# Autodesk Inventor assembly: PeltierController
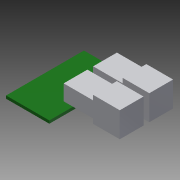
[picture p0: Inventor's stored thumbnail of the model, 180x180]
Saved by Autodesk Inventor 2014 (Build 180170000, 170)
## iProperties
Created: 2015-04-19
Part Number: PeltierController
Document SubType Name: Assembly
Designer: Owner
Author: Owner
## Documents named in this file (4)
- C:\Users\Owner\Documents\APC\FrontEnd\IAM\Common\PeltierController.iam
- C:\Users\Owner\Documents\APC\FrontEnd\IAM\Common\PeltierControllerBoard.ipt
- C:\Users\Owner\Documents\APC\FrontEnd\IAM\Common\TE_2Pin.ipt
- C:\Users\Owner\Documents\APC\FrontEnd\IAM\Common\TE_2Pin_Male.ipt
## Components (5 placed, 3 different names)
1. PeltierControllerBoard:1 — Mate:1, Mate:2, Flush:1, Flush:2, Flush:3, Flush:4
2. TE_2Pin:1 — Mate:1, Flush:2, Flush:3, Mate:3, Mate:6, Flush:6
3. TE_2Pin:2 — Mate:2, Flush:1, Flush:4, Mate:4, Mate:5, Flush:5
4. TE_2Pin_Male:1 — Mate:4, Mate:5, Flush:5
5. TE_2Pin_Male:2 — Mate:3, Mate:6, Flush:6
## Relationships (12: Mate 6, Flush 6)
- Mate:1: PeltierControllerBoard:1 ↔ TE_2Pin:1
- Mate:2: PeltierControllerBoard:1 ↔ TE_2Pin:2
- Flush:1 (19.8679 mm): PeltierControllerBoard:1 ↔ TE_2Pin:2
- Flush:2 (-19.8679 mm): PeltierControllerBoard:1 ↔ TE_2Pin:1
- Flush:3 (0.4953 mm): PeltierControllerBoard:1 ↔ TE_2Pin:1
- Flush:4 (17.8206 mm): PeltierControllerBoard:1 ↔ TE_2Pin:2
- Mate:3: TE_2Pin:1 ↔ TE_2Pin_Male:2
- Mate:4: TE_2Pin:2 ↔ TE_2Pin_Male:1
- Mate:5: TE_2Pin:2 ↔ TE_2Pin_Male:1
- Mate:6: TE_2Pin:1 ↔ TE_2Pin_Male:2
- Flush:5: TE_2Pin:2 ↔ TE_2Pin_Male:1
- Flush:6: TE_2Pin:1 ↔ TE_2Pin_Male:2
